# Autodesk Inventor assembly: printer
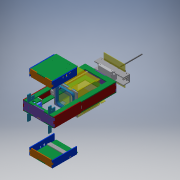
[picture p0: Inventor's stored thumbnail of the model, 180x180]
Saved by Autodesk Inventor 2019 (Build 230136000, 136)
## iProperties
Created: 2015-03-06
Part Number: printer
Document SubType Name: Assembly
Designer: cruiser
Author: cruiser
## Documents named in this file (15)
- C:\Users\cruiser\Desktop\models\3d printers\laserresin3\printer.iam
- C:\Users\cruiser\Desktop\models\3d printers\laserresin3\nema17.ipt
- C:\Users\cruiser\Desktop\models\3d printers\laserresin3\shf8.ipt
- C:\Users\cruiser\Desktop\models\3d printers\laserresin3\m8_rail.ipt
- C:\Users\cruiser\Desktop\models\3d printers\laserresin3\threaded_rod.ipt
- C:\Users\cruiser\Desktop\models\3d printers\laserresin3\door.ipt
- C:\Users\cruiser\Desktop\models\3d printers\laserresin3\frame2.ipt
- C:\Users\cruiser\Desktop\models\3d printers\laserresin3\carrier2.ipt
- C:\Users\cruiser\Desktop\models\3d printers\laserresin3\drawer.ipt
- C:\Users\cruiser\Desktop\models\3d printers\laserresin3\crane3.ipt
- C:\Users\cruiser\Desktop\models\3d printers\laserresin3\lmk8luu.ipt
- C:\Users\cruiser\Desktop\models\3d printers\laserresin3\bedsm.ipt
- C:\Users\cruiser\Desktop\models\3d printers\laserresin3\inner_tray.ipt
- C:\Users\cruiser\Desktop\models\3d printers\laserresin3\inner_tray_bottom.ipt
- C:\Users\cruiser\Desktop\models\3d printers\laserresin3\laser.ipt
## Components (19 placed, 14 different names)
1. frame2:1 — Flush:5, Mate:59, Mate:60, Flush:6, Mate:67, Flush:7, Mate:68, Mate:92, Mate:93, Mate:94, Mate:95, Mate:119, Mate:124, Flush:126
2. carrier2:1 — Flush:5, Mate:59, Mate:60, Mate:61, Mate:62, Mate:63, Mate:64, Mate:65, Mate:66, Mate:87, Mate:88, Mate:115, Mate:116, Mate:117, Mate:118, Mate:120, Mate:123
3. shf8:5 — Mate:61, Mate:62, Mate:63
4. shf8:6 — Mate:64, Mate:65, Mate:66
5. m8_rail:3 — Flush:6, Mate:67, Mate:108
6. m8_rail:4 — Flush:7, Mate:68, Mate:107
7. nema17:2 — Mate:81, Mate:82, Mate:98, Mate:99, Mate:100
8. threaded_rod:4 — Mate:81, Mate:82
9. door:3 — Mate:87, Mate:88, Mate:118
10. door:4 — Mate:120, Mate:123
11. drawer:1 — Mate:92, Mate:93, Mate:119
12. drawer:2 — Mate:94, Mate:95
13. crane3:1 — Mate:98, Mate:99, Mate:100, Mate:101, Mate:102, Mate:103, Mate:104, Mate:105, Mate:106, Mate:109, Mate:110, Mate:111
14. lmk8luu:1 — Mate:101, Mate:102, Mate:103, Mate:108
15. lmk8luu:2 — Mate:104, Mate:105, Mate:106, Mate:107
16. bedsm:1 — Mate:109, Mate:110, Mate:111
17. inner_tray:1 — Mate:112, Mate:113, Mate:114, Mate:115, Mate:116, Mate:117
18. inner_tray_bottom:1 — Mate:112, Mate:113, Mate:114
19. laser:1 — Mate:124, Flush:126
## Relationships (47: Mate 43, Flush 4)
- Flush:5: frame2:1 ↔ carrier2:1
- Mate:59: frame2:1 ↔ carrier2:1
- Mate:60: frame2:1 ↔ carrier2:1
- Mate:61: carrier2:1 ↔ shf8:5
- Mate:62: carrier2:1 ↔ shf8:5
- Mate:63: carrier2:1 ↔ shf8:5
- Mate:64: carrier2:1 ↔ shf8:6
- Mate:65: carrier2:1 ↔ shf8:6
- Mate:66: carrier2:1 ↔ shf8:6
- Flush:6: frame2:1 ↔ m8_rail:3
- Mate:67: frame2:1 ↔ m8_rail:3
- Flush:7: frame2:1 ↔ m8_rail:4
- Mate:68: frame2:1 ↔ m8_rail:4
- Mate:81: nema17:2 ↔ threaded_rod:4
- Mate:82: nema17:2 ↔ threaded_rod:4
- Mate:87: carrier2:1 ↔ door:3
- Mate:88: carrier2:1 ↔ door:3
- Mate:92: frame2:1 ↔ drawer:1
- Mate:93: frame2:1 ↔ drawer:1
- Mate:94: frame2:1 ↔ drawer:2
- Mate:95: frame2:1 ↔ drawer:2
- Mate:98: nema17:2 ↔ crane3:1
- Mate:99: nema17:2 ↔ crane3:1
- Mate:100: nema17:2 ↔ crane3:1
- Mate:101: crane3:1 ↔ lmk8luu:1
- Mate:102: crane3:1 ↔ lmk8luu:1
- Mate:103: crane3:1 ↔ lmk8luu:1
- Mate:104: crane3:1 ↔ lmk8luu:2
- Mate:105: crane3:1 ↔ lmk8luu:2
- Mate:106: crane3:1 ↔ lmk8luu:2
- Mate:107: m8_rail:4 ↔ lmk8luu:2
- Mate:108: m8_rail:3 ↔ lmk8luu:1
- Mate:109: crane3:1 ↔ bedsm:1
- Mate:110: crane3:1 ↔ bedsm:1
- Mate:111 (0.3 mm): crane3:1 ↔ bedsm:1
- Mate:112: inner_tray:1 ↔ inner_tray_bottom:1
- Mate:113: inner_tray:1 ↔ inner_tray_bottom:1
- Mate:114: inner_tray:1 ↔ inner_tray_bottom:1
- Mate:115: carrier2:1 ↔ inner_tray:1
- Mate:116: carrier2:1 ↔ inner_tray:1
- Mate:117: carrier2:1 ↔ inner_tray:1
- Mate:118: carrier2:1 ↔ door:3
- Mate:119: frame2:1 ↔ drawer:1
- Mate:120: carrier2:1 ↔ door:4
- Mate:123: carrier2:1 ↔ door:4
- Mate:124: frame2:1 ↔ laser:1
- Flush:126: frame2:1 ↔ laser:1
